# Autodesk Inventor assembly: Assembly_singleLeg
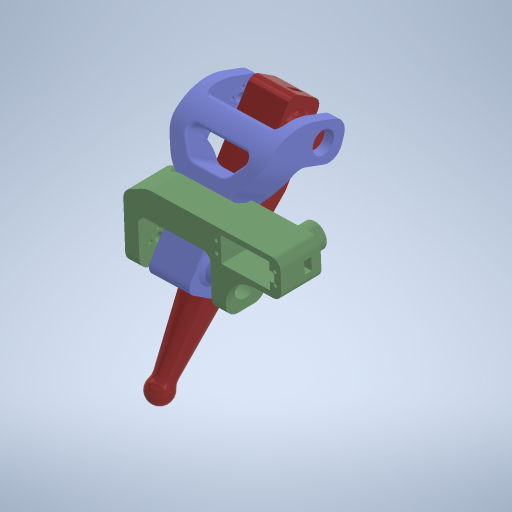
[picture p0: Inventor's stored thumbnail of the model, 512x512]
Saved by Autodesk Inventor 2023 (Build 270158000, 158)
## iProperties
Created: 2023-11-24
Part Number: Assembly_singleLeg
Document SubType Name: Assembly
Designer: Dawid
Author: Dawid
## Documents named in this file (4)
- C:\Users\Dawid\Desktop\Robot\Github\DogRobot_MyEngineeringWork\3D_element\Assembly_singleLeg.iam
- C:\Users\Dawid\Desktop\Robot\Github\DogRobot_MyEngineeringWork\3D_element\Leg1_1.ipt
- C:\Users\Dawid\Desktop\Robot\Github\DogRobot_MyEngineeringWork\3D_element\Leg1_2.ipt
- C:\Users\Dawid\Desktop\Robot\Github\DogRobot_MyEngineeringWork\3D_element\Leg1_3.ipt
## Components (3 placed, 3 different names)
1. Leg1_1:1 — Rotational:2
2. Leg1_2:1 — Rotational:2, Rotational:5
3. Leg1_3:1 — Rotational:5
## Relationships (2: RevoluteJoint 2)
- Rotational:2 [RevoluteJoint]: Leg1_1:1 ↔ Leg1_2:1
- Rotational:5 [RevoluteJoint]: Leg1_2:1 ↔ Leg1_3:1
